# Autodesk Inventor assembly: bumper
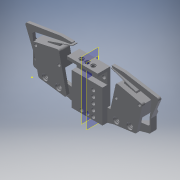
[picture p0: Inventor's stored thumbnail of the model, 180x180]
Saved by Autodesk Inventor 2016 (Build 200138000, 138)
## iProperties
Created: 2016-02-16
Part Number: bumper
Document SubType Name: Assembly
Designer: jforce
Author: jforce
## Documents named in this file (6)
- C:\Users\jforce\Dropbox\gmu\ece590\robot_models\bumper.iam
- C:\Users\jforce\Dropbox\gmu\ece590\robot_models\bumper_plate.ipt
- C:\Users\jforce\Dropbox\gmu\ece590\robot_models\switch.ipt
- C:\Users\jforce\Dropbox\gmu\ece590\robot_models\bump_switch_mount.ipt
- C:\Users\jforce\Dropbox\gmu\ece590\robot_models\switch_MIR1.ipt
- C:\Users\jforce\Dropbox\gmu\ece590\robot_models\bump_switch_mount_MIR2.ipt
## Components (5 placed, 5 different names)
1. bumper_plate:1 — Mate:2, Angle:1
2. switch:1 — Flush:1, Mate:1
3. bump_switch_mount:1 — Flush:1, Mate:1
4. switch_MIR1:1
5. bump_switch_mount_MIR2:1
## Relationships (4: Mate 2, Flush 1, Angle 1)
- Flush:1: switch:1 ↔ bump_switch_mount:1
- Mate:1: switch:1 ↔ bump_switch_mount:1
- Mate:2: bumper_plate:1
- Angle:1 (0 deg): bumper_plate:1
